# Autodesk Inventor assembly: Teensy3.1
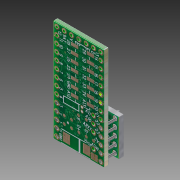
[picture p0: Inventor's stored thumbnail of the model, 180x180]
Saved by Autodesk Inventor 2014 (Build 180170000, 170)
## iProperties
Created: 2014-04-23
Part Number: Teensy3.1
Document SubType Name: Assembly
Designer: larraguetajunior
Description: Teensy3.1
Mass: 3 g
Surface Area: 27.9252 cm^2
Volume: 1.41306 cm^3
Author: larraguetajunior
## Documents named in this file (6)
- C:\Users\jose\Dropbox\UAV\- AIRDATACOMPUTER\commerciali\TEENSY3.1\Teensy3.1.iam
- C:\Users\jose\Dropbox\UAV\- AIRDATACOMPUTER\commerciali\TEENSY3.1\Teensyboard.ipt
- C:\Users\jose\Dropbox\UAV\- AIRDATACOMPUTER\commerciali\TEENSY3.1\MiniUSB.ipt
- C:\Users\jose\Dropbox\UAV\- AIRDATACOMPUTER\commerciali\MICRO SD ADAPTER\microsdadapterboard.ipt
- C:\Users\jose\Dropbox\UAV\- AIRDATACOMPUTER\commerciali\MICRO SD ADAPTER\5031821852MICROSDADAPTER.ipt
- C:\Users\jose\Dropbox\UAV\- AIRDATACOMPUTER\commerciali\MICRO SD ADAPTER\pinSDCARDTOTEENSY.ipt
## Components (14 placed, 5 different names)
1. 101 Teensyboard:1 — Allineato:3, Allineato:2, Coincidente:3, Coincidente:4, Coincidente:5, Allineato:4, Mate:6, Mate:7
2. MiniUSB:1 — Coincidente:3, Coincidente:4, Coincidente:5, Mate:8
3. microsdadapterboard:1 — Mate:6, Mate:7, Mate:8, Mate:9, Mate:10, Flush:5
4. 5031821852MICROSDADAPTER:1 — Mate:9
5. pinSDCARDTOTEENSY:1 — Mate:10, Flush:5
6. pinSDCARDTOTEENSY:2
7. pinSDCARDTOTEENSY:3
8. pinSDCARDTOTEENSY:4
9. pinSDCARDTOTEENSY:5
10. pinSDCARDTOTEENSY:6
11. pinSDCARDTOTEENSY:7
12. pinSDCARDTOTEENSY:8
13. pinSDCARDTOTEENSY:9
14. pinSDCARDTOTEENSY:10
## Component patterns: (10 elements, first: pinSDCARDTOTEENSY:1)
## Relationships (12: Mate 8, Flush 4)
- Allineato:3 [Flush]: 101 Teensyboard:1
- Allineato:2 [Flush]: 101 Teensyboard:1
- Coincidente:3 [Mate]: 101 Teensyboard:1 ↔ MiniUSB:1
- Coincidente:4 [Mate]: 101 Teensyboard:1 ↔ MiniUSB:1
- Coincidente:5 [Mate] (1.5 mm): 101 Teensyboard:1 ↔ MiniUSB:1
- Allineato:4 [Flush]: 101 Teensyboard:1
- Mate:6: 101 Teensyboard:1 ↔ microsdadapterboard:1
- Mate:7: 101 Teensyboard:1 ↔ microsdadapterboard:1
- Mate:8 (1 mm): MiniUSB:1 ↔ microsdadapterboard:1
- Mate:9: microsdadapterboard:1 ↔ 5031821852MICROSDADAPTER:1
- Mate:10: microsdadapterboard:1 ↔ pinSDCARDTOTEENSY:1
- Flush:5: microsdadapterboard:1 ↔ pinSDCARDTOTEENSY:1
